# Autodesk Inventor assembly: E-AXIS ASSEMBLY P2.0
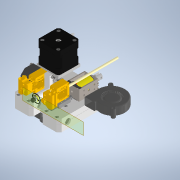
[picture p0: Inventor's stored thumbnail of the model, 180x180]
Saved by Autodesk Inventor 2020.3 (Build 243373010, 373A)
## iProperties
Created: 2019-12-19
Part Number: E-AXIS ASSEMBLY P2.0
Document SubType Name: Assembly
Designer: pepd9
Mass: 917.379 g
Surface Area: 2479.59 cm^2
Volume: 339.663 cm^3
Density: 2.70085 g/cm^3
Author: pepd9
## Documents named in this file (19)
- D:\Designs\MK3PRO P1\E-Axis\E-AXIS ASSEMBLY P2.1.iam
- D:\Designs\MK3PRO P1\COMPONENTS\LM10UU.ipt
- D:\Designs\MK3PRO P1\E-Axis\PINDA_Probe.ipt
- D:\Designs\MK3PRO P1\COMPONENTS\Bondtech Driver.ipt
- D:\Designs\MK3PRO P1\COMPONENTS\FAN_5015_BLOWER.ipt
- D:\Designs\MK3PRO P1\E-Axis\V2 - Dual Extruder\mosquito_model_to_publish.ipt
- D:\Designs\MK3PRO P1\COMPONENTS\625 Bearing.ipt
- D:\Designs\MK3PRO P1\E-Axis\V2 - Dual Extruder\Carriage Mount V2.1.ipt
- D:\Designs\MK3PRO P1\E-Axis\V2 - Dual Extruder\Carriage Backplate.ipt
- D:\Designs\MK3PRO P1\E-Axis\V2 - Dual Extruder\Extruder Backplate V2.1.ipt
- D:\Designs\MK3PRO P1\E-Axis\Motor Mount V2.1.ipt
- D:\Designs\MK3PRO P1\COMPONENTS\TW-04-07.ipt
- D:\Designs\MK3PRO P1\COMPONENTS\TS-04-07-100.ipt
- D:\Designs\MK3PRO P1\E-Axis\E-AXIS ASSEMBLY P2.0\Design Accelerator\Bolted Connection1.iam
- D:\Designs\MK3PRO P1\E-Axis\E-AXIS ASSEMBLY P2.0\Design Accelerator\Bolted Connection2.iam
- D:\Designs\MK3PRO P1\E-Axis\Extruder_stepper_motor V2.iam
- D:\Designs\MK3PRO P1\COMPONENTS\MF25150V1-1000U-A99.ipt
- D:\Designs\MK3PRO P1\E2\Solenoid Assembly.iam
- D:\Designs\MK3PRO P1\E-Axis\E2 Teflon.ipt
## Components (22 placed, 17 different names)
1. LM10UU:1 — Mate:47, Mate:48, Mate:53, Mate:57, Mate:58, Mate:59, Mate:60
2. LM10UU:2 — Mate:49, Mate:50
3. LM10UU:3 — Mate:50, Mate:51, Mate:52, Flush:6, Mate:61
4. mosquito_model_to_publish:1 — Mate:42, Mate:63, Mate:92, Flush:20
5. mosquito_model_to_publish:2 — Mate:41, Flush:12, Mate:65, Mate:71, Mate:79, Mate:86, Mate:87, Mate:88
6. Extruder_stepper_motor V2:1 [sub-assembly] — Mate:54, Flush:11, Mate:83, Mate:84
7. Bondtech Driver:1 — Mate:54, Mate:77, Mate:78, Mate:79
8. PINDA_Probe:1 — Mate:55, Mate:56
9. Carriage Mount V2.1:1 — Mate:57, Mate:58, Mate:62, Flush:9, Flush:10, Mate:69, Flush:14, Mate:74, Mate:82, Mate:84, Mate:93
10. Carriage Backplate:1 — Mate:59, Mate:60, Mate:61, Mate:67, Mate:68, Mate:70, Flush:13
11. Extruder Backplate V2.1:1 — Mate:62, Flush:9, Flush:10, Mate:65
12. Motor Mount V2.1:1 — Flush:11
13. TW-04-07:1 — Mate:72, Mate:73, Flush:15, Mate:92
14. TS-04-07-100:1 — Mate:72, Mate:73, Flush:15, Mate:74
15. Bolted Connection:1 [sub-assembly] — Mate:67, Mate:68, Mate:69
16. FAN_5015_BLOWER:1 — Mate:70, Flush:13
17. FAN_5015_BLOWER:2 — Mate:71, Flush:14
18. 625 Bearing:1 — Mate:82, Mate:83
19. MF25150V1-1000U-A99:1 — Mate:86, Mate:87, Mate:88, Mate:89, Mate:90
20. Bolted Connection:2 [sub-assembly] — Mate:89, Mate:90
21. Solenoid Assembly:1 [sub-assembly] — Mate:93
22. E2 Teflon:1 — Flush:20
## Relationships (58: Mate 41, Flush 17)
- Flush:1 (30 mm)
- Flush:2 (-4.4 mm)
- Mate:41: mosquito_model_to_publish:2
- Mate:42: mosquito_model_to_publish:1
- Mate:47: LM10UU:1
- Mate:48 (-14.5 mm): LM10UU:1
- Mate:49 (14 mm): LM10UU:2
- Mate:50: LM10UU:2 ↔ LM10UU:3
- Mate:51: LM10UU:3
- Flush:4 (25 mm)
- Flush:5 (55 mm)
- Mate:52: LM10UU:3
- Mate:53: LM10UU:1
- Flush:6 (14 mm): LM10UU:3
- Mate:54: Extruder_stepper_motor V2:1 ↔ Bondtech Driver:1
- Flush:8 (10 mm)
- Mate:55 (1 mm): PINDA_Probe:1
- Mate:56: PINDA_Probe:1
- Mate:57: LM10UU:1 ↔ Carriage Mount V2.1:1
- Mate:58: LM10UU:1 ↔ Carriage Mount V2.1:1
- Mate:59: LM10UU:1 ↔ Carriage Backplate:1
- Mate:60: LM10UU:1 ↔ Carriage Backplate:1
- Mate:61: LM10UU:3 ↔ Carriage Backplate:1
- Mate:62: Carriage Mount V2.1:1 ↔ Extruder Backplate V2.1:1
- Flush:9: Carriage Mount V2.1:1 ↔ Extruder Backplate V2.1:1
- Flush:10: Carriage Mount V2.1:1 ↔ Extruder Backplate V2.1:1
- Flush:11: Extruder_stepper_motor V2:1 ↔ Motor Mount V2.1:1
- Mate:63 (15 mm): mosquito_model_to_publish:1
- Flush:12 (15 mm): mosquito_model_to_publish:2
- Mate:65 (2 mm): mosquito_model_to_publish:2 ↔ Extruder Backplate V2.1:1
- Mate:67: Carriage Backplate:1 ↔ Bolted Connection:1
- Mate:68: Carriage Backplate:1 ↔ Bolted Connection:1
- Mate:69: Carriage Mount V2.1:1 ↔ Bolted Connection:1
- Mate:70: Carriage Backplate:1 ↔ FAN_5015_BLOWER:1
- Flush:13: Carriage Backplate:1 ↔ FAN_5015_BLOWER:1
- Mate:71: mosquito_model_to_publish:2 ↔ FAN_5015_BLOWER:2
- Flush:14: Carriage Mount V2.1:1 ↔ FAN_5015_BLOWER:2
- Mate:72: TW-04-07:1 ↔ TS-04-07-100:1
- Mate:73: TW-04-07:1 ↔ TS-04-07-100:1
- Flush:15: TW-04-07:1 ↔ TS-04-07-100:1
- Mate:74: Carriage Mount V2.1:1 ↔ TS-04-07-100:1
- Flush:17 (30.5 mm)
- Mate:77 (1.2 mm): Bondtech Driver:1
- Flush:18 (-21.5 mm)
- Flush:19 (4 mm)
- Mate:78: Bondtech Driver:1
- Mate:79 (22 mm): mosquito_model_to_publish:2 ↔ Bondtech Driver:1
- Mate:82: Carriage Mount V2.1:1 ↔ 625 Bearing:1
- Mate:83: Extruder_stepper_motor V2:1 ↔ 625 Bearing:1
- Mate:84 (0.5 mm): Extruder_stepper_motor V2:1 ↔ Carriage Mount V2.1:1
- Mate:86: mosquito_model_to_publish:2 ↔ MF25150V1-1000U-A99:1
- Mate:87: mosquito_model_to_publish:2 ↔ MF25150V1-1000U-A99:1
- Mate:88: mosquito_model_to_publish:2 ↔ MF25150V1-1000U-A99:1
- Mate:89: MF25150V1-1000U-A99:1 ↔ Bolted Connection:2
- Mate:90: MF25150V1-1000U-A99:1 ↔ Bolted Connection:2
- Mate:92 (4 mm): mosquito_model_to_publish:1 ↔ TW-04-07:1
- Mate:93: Carriage Mount V2.1:1 ↔ Solenoid Assembly:1
- Flush:20: mosquito_model_to_publish:1 ↔ E2 Teflon:1
## Named parameters: Rod_Spacing = 55 mm, Bearing_Spacing = 28 mm
